# Autodesk Inventor assembly: gimbal_servo
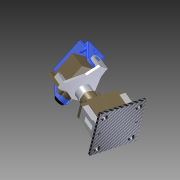
[picture p0: Inventor's stored thumbnail of the model, 180x180]
Saved by Autodesk Inventor 2015 SP1 (Build 190203100, 203)
## iProperties
Created: 2015-07-09
Part Number: gimbal_servo
Document SubType Name: Assembly
Designer: Alexandre Cherpillod
Mass: 35.7877 g
Surface Area: 162.355 cm^2
Volume: 24.1959 cm^3
Density: 1.47908 g/cm^3
Author: Alexandre Cherpillod
## Documents named in this file (8)
- D:\_windows\_github_doc\MAVRIC\Mechanics\myCopter_CAD\Inventor\Gimbal_Servo\gimbal_servo.iam
- D:\_windows\_github_doc\MAVRIC\Mechanics\myCopter_CAD\Inventor\Gimbal_Servo\servo_FatShark_180MG.ipt
- D:\_windows\_github_doc\MAVRIC\Mechanics\myCopter_CAD\Inventor\Gimbal_Servo\shaft_nut_for_FatShark_180MG.ipt
- D:\_windows\_github_doc\MAVRIC\Mechanics\myCopter_CAD\Inventor\Gimbal_Servo\servo_gimbal_interpart_1.ipt
- D:\_windows\_github_doc\MAVRIC\Mechanics\myCopter_CAD\Inventor\Gimbal_Servo\servo_nut_2_for_FatShark_180MG.ipt
- D:\_windows\_github_doc\MAVRIC\Mechanics\myCopter_CAD\Inventor\Gimbal_Servo\servo_camera_fix_for_FatShark_180MG.ipt
- D:\_windows\_github_doc\MAVRIC\Mechanics\myCopter_CAD\Inventor\Gimbal_Servo\servo_attachement.ipt
- D:\_windows\_github_doc\MAVRIC\Mechanics\myCopter_CAD\Inventor\Gimbal_Servo\carbon_bump_servo.ipt
## Components (9 placed, 7 different names)
1. servo_FatShark_180MG:1 — Mate:1, Flush:1, Mate:10, Mate:11, Angle:2, Mate:12, Angle:3, Mate:17
2. shaft_nut_for_FatShark_180MG:1 — Mate:1, Flush:1, Mate:2, Mate:3, Mate:4
3. servo_gimbal_interpart_1:1 — Mate:2, Mate:3, Mate:4, Insert:1, Angle:1, Mate:7
4. servo_FatShark_180MG:2 — Mate:5, Mate:8, Insert:1, Angle:1
5. servo_nut_2_for_FatShark_180MG:1 — Mate:5, Mate:8, Mate:9
6. servo_camera_fix_for_FatShark_180MG:1 — Mate:7, Mate:9
7. carbon_bump_servo:1 — Mate:14, Mate:15, Mate:16
8. servo_attachement:1 — Mate:10, Mate:11, Angle:2, Mate:14
9. servo_attachement:2 — Mate:12, Angle:3, Mate:15, Mate:16, Mate:17
## Relationships (20: Mate 15, Angle 3, Flush 1, Insert 1)
- Mate:1: servo_FatShark_180MG:1 ↔ shaft_nut_for_FatShark_180MG:1
- Flush:1 (-5 mm): servo_FatShark_180MG:1 ↔ shaft_nut_for_FatShark_180MG:1
- Mate:2: shaft_nut_for_FatShark_180MG:1 ↔ servo_gimbal_interpart_1:1
- Mate:3: shaft_nut_for_FatShark_180MG:1 ↔ servo_gimbal_interpart_1:1
- Mate:4: shaft_nut_for_FatShark_180MG:1 ↔ servo_gimbal_interpart_1:1
- Mate:5: servo_FatShark_180MG:2 ↔ servo_nut_2_for_FatShark_180MG:1
- Mate:8 (3.9 mm): servo_FatShark_180MG:2 ↔ servo_nut_2_for_FatShark_180MG:1
- Insert:1 (-2.5 mm): servo_gimbal_interpart_1:1 ↔ servo_FatShark_180MG:2
- Angle:1 (180 deg): servo_gimbal_interpart_1:1 ↔ servo_FatShark_180MG:2
- Mate:7: servo_gimbal_interpart_1:1 ↔ servo_camera_fix_for_FatShark_180MG:1
- Mate:9: servo_nut_2_for_FatShark_180MG:1 ↔ servo_camera_fix_for_FatShark_180MG:1
- Mate:10: servo_FatShark_180MG:1 ↔ servo_attachement:1
- Mate:11: servo_FatShark_180MG:1 ↔ servo_attachement:1
- Angle:2 (0 deg): servo_FatShark_180MG:1 ↔ servo_attachement:1
- Mate:12: servo_FatShark_180MG:1 ↔ servo_attachement:2
- Angle:3 (180 deg): servo_FatShark_180MG:1 ↔ servo_attachement:2
- Mate:14: carbon_bump_servo:1 ↔ servo_attachement:1
- Mate:15: carbon_bump_servo:1 ↔ servo_attachement:2
- Mate:16: carbon_bump_servo:1 ↔ servo_attachement:2
- Mate:17: servo_FatShark_180MG:1 ↔ servo_attachement:2
